# Autodesk Inventor assembly: FANUCs430
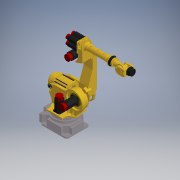
[picture p0: Inventor's stored thumbnail of the model, 180x180]
Saved by Autodesk Inventor 2017 (Build 210142000, 142)
## iProperties
Created: 2002-03-22
Part Number: FANUCs430
Document SubType Name: Assembly
Designer: sdotson
Control State: 0
Master: False
Checked Out: False
Shininess: 0.0
Length Units: 11269
Angle Units: 11279
Time Units: 11290
Mass Units: 11283
Length Display Precision: 3
Angle Display Precision: 2
Compacted: True
Density: 0.0
Volumn: 0.0
Area: 0.0
PropertySet Name: Model Information
Author: sdotson
## Documents named in this file (36)
- C:\Users\diego\Desktop\Example Inventor\12\toExporti.iam
- C:\Users\diego\Desktop\Example Inventor\12\s430if1.ipt
- C:\Users\diego\Desktop\Example Inventor\12\s430if13.ipt
- C:\Users\diego\Desktop\Example Inventor\12\s430if12.ipt
- C:\Users\diego\Desktop\Example Inventor\12\s430if10.ipt
- C:\Users\diego\Desktop\Example Inventor\12\s430if9.ipt
- C:\Users\diego\Desktop\Example Inventor\12\s430if14.ipt
- C:\Users\diego\Desktop\Example Inventor\12\s430if86.ipt
- C:\Users\diego\Desktop\Example Inventor\12\s430if85.ipt
- C:\Users\diego\Desktop\Example Inventor\12\s430if87.ipt
- C:\Users\diego\Desktop\Example Inventor\12\s430if88.ipt
- C:\Users\diego\Desktop\Example Inventor\12\s430if82.ipt
- C:\Users\diego\Desktop\Example Inventor\12\s430if83.ipt
- C:\Users\diego\Desktop\Example Inventor\12\s430if84.ipt
- C:\Users\diego\Desktop\Example Inventor\12\s430if34.ipt
- C:\Users\diego\Desktop\Example Inventor\12\s430if40.ipt
- C:\Users\diego\Desktop\Example Inventor\12\s430if63.ipt
- C:\Users\diego\Desktop\Example Inventor\12\NutPlate.iam
- C:\Users\diego\Desktop\Example Inventor\12\s430if24.ipt
- C:\Users\diego\Desktop\Example Inventor\12\NutPlate2.iam
- C:\Users\diego\Desktop\Example Inventor\12\s430if30.ipt
- C:\Users\diego\Desktop\Example Inventor\12\s430if31.ipt
- C:\Users\diego\Desktop\Example Inventor\12\s430if58.ipt
- C:\Users\diego\Desktop\Example Inventor\12\s430if57.ipt
- C:\Users\diego\Desktop\Example Inventor\12\s430if35.ipt
- C:\Users\diego\Desktop\Example Inventor\12\s430if59.ipt
- C:\Users\diego\Desktop\Example Inventor\12\s430if15.ipt
- C:\Users\diego\Desktop\Example Inventor\12\s430if74.ipt
- C:\Users\diego\Desktop\Example Inventor\12\SmallServo.iam
- C:\Users\diego\Desktop\Example Inventor\12\s430if23.ipt
- C:\Users\diego\Desktop\Example Inventor\12\s430if3.ipt
- C:\Users\diego\Desktop\Example Inventor\12\s430if22.ipt
- C:\Users\diego\Desktop\Example Inventor\12\s430if5.ipt
- C:\Users\diego\Desktop\Example Inventor\12\s430if6.ipt
- C:\Users\diego\Desktop\Example Inventor\12\AXIS5.ipt
- C:\Users\diego\Desktop\Example Inventor\12\AXIS6.ipt
## Components (50 placed, 35 different names)
1. s430if1:1 — Insertar:1, Ángulo:2, Nivelación:11, Nivelación:12, Coincidencia:37, Ángulo:13
2. s430if13:1 — Insertar:1, Insertar:2
3. s430if12:1 — Insertar:2, Insertar:3
4. s430if12:2 — Insertar:3, Insertar:4
5. s430if10:1 — Insertar:4, Insertar:5
6. s430if9:1 — Insertar:5, Coincidencia:1, Coincidencia:2
7. J1 — Coincidencia:1, Coincidencia:2, Coincidencia:3, Nivelación:1, Coincidencia:4, Insertar:6, Insertar:15, Insertar:16, Coincidencia:16, Insertar:17, Insertar:18, Coincidencia:17, Coincidencia:18, Insertar:19, Coincidencia:19, Coincidencia:20, Nivelación:3, Insertar:22, Ángulo:12
8. s430if86:1 — Coincidencia:3, Nivelación:1, Coincidencia:4, Nivelación:2, Coincidencia:5, Coincidencia:6
9. s430if85:1 — Nivelación:2, Coincidencia:5, Coincidencia:6, Coincidencia:7, Coincidencia:8, Ángulo:1
10. s430if87:1 — Coincidencia:7, Coincidencia:8, Ángulo:1
11. s430if88:1 — Coincidencia:12, Coincidencia:14, Ángulo:4
12. s430if82:1 — Coincidencia:11, Coincidencia:13, Coincidencia:14, Ángulo:3, Ángulo:4
13. s430if83:1 — Coincidencia:9, Coincidencia:10, Ángulo:2, Coincidencia:11, Coincidencia:12, Coincidencia:13, Ángulo:3
14. s430if84:1 — Insertar:6, Coincidencia:9, Coincidencia:10
15. s430if34:1 — Insertar:7, Insertar:8, Insertar:9, Insertar:10, Insertar:11, Insertar:12, Insertar:13, Insertar:14, Coincidencia:15, Coincidencia:16, Ángulo:11, Coincidencia:38
16. s430if40:1 — Insertar:7
17. s430if40:2 — Insertar:8
18. s430if40:3 — Insertar:10
19. s430if40:4 — Insertar:9
20. s430if40:5 — Insertar:11
21. s430if40:6 — Insertar:12
22. s430if40:7 — Insertar:13
23. s430if40:8 — Insertar:14
24. s430if63:1 — Insertar:15, Coincidencia:15
25. s430if63:2 — Insertar:16
26. NutPlate:1 [sub-assembly] — Insertar:18
27. NutPlate:2 [sub-assembly] — Insertar:17
28. J2 — Coincidencia:17, Coincidencia:18, Coincidencia:24, Insertar:23, Insertar:24, Ángulo:13, Ángulo:14
29. NutPlate2:1 [sub-assembly] — Insertar:19
30. s430if30:1 — Coincidencia:19, Coincidencia:20, Nivelación:3, Coincidencia:21, Coincidencia:22
31. s430if31:1 — Coincidencia:21, Coincidencia:22
32. s430if58:1 — Coincidencia:23, Insertar:21, Coincidencia:24
33. s430if57:1 — Coincidencia:23, Insertar:20, Insertar:21
34. s430if35:1 — Insertar:20, Ángulo:11, Coincidencia:38
35. s430if59:1 — Insertar:22
36. J3 — Insertar:23, Coincidencia:25, Coincidencia:26, Ángulo:5, Coincidencia:27, Coincidencia:29, Coincidencia:31, Nivelación:4, Nivelación:5, Coincidencia:32, Coincidencia:33, Nivelación:8, Nivelación:9, Insertar:25, Ángulo:10, Ángulo:14
37. s430if74:1 — Insertar:24
38. s430if86:2 — Coincidencia:25, Coincidencia:26, Ángulo:5, Coincidencia:28, Ángulo:7
39. s430if85:2 — Coincidencia:27, Coincidencia:28, Coincidencia:30, Ángulo:6, Ángulo:7
40. s430if87:2 — Coincidencia:29, Coincidencia:30, Ángulo:6
41. SmallServo:1 [sub-assembly] — Coincidencia:31, Nivelación:4, Nivelación:5, Ángulo:8, Nivelación:7
42. SmallServo:2 [sub-assembly] — Coincidencia:32, Ángulo:8, Ángulo:9, Nivelación:6, Nivelación:7, Nivelación:8
43. SmallServo:3 [sub-assembly] — Coincidencia:33, Ángulo:9, Nivelación:6, Nivelación:9
44. s430if23:1 — Insertar:25, Ángulo:10, Insertar:26, Ángulo:15
45. s430if3:1 — Insertar:26, Insertar:27
46. J4 — Insertar:27, Coincidencia:34, Coincidencia:35, Coincidencia:36, Nivelación:10, Ángulo:15, Ángulo:16
47. s430if5:1 — Coincidencia:34, Insertar:28, Insertar:29
48. s430if6:1 — Coincidencia:35, Insertar:29
49. J5 — Coincidencia:36, Nivelación:10, Insertar:28, Insertar:30, Angle, Ángulo:16
50. J6 — Insertar:30, Angle
## Relationships (97: Mate 38, Insert 30, Angle 17, Flush 12)
- Insertar:1: s430if1:1 ↔ s430if13:1
- Insertar:2: s430if13:1 ↔ s430if12:1
- Insertar:3: s430if12:1 ↔ s430if12:2
- Insertar:4: s430if12:2 ↔ s430if10:1
- Insertar:5: s430if10:1 ↔ s430if9:1
- Coincidencia:1 [Mate]: s430if9:1 ↔ J1
- Coincidencia:2 [Mate]: s430if9:1 ↔ J1
- Coincidencia:3 [Mate]: J1 ↔ s430if86:1
- Nivelación:1 [Flush] (117.314 mm): J1 ↔ s430if86:1
- Coincidencia:4 [Mate]: J1 ↔ s430if86:1
- Nivelación:2 [Flush]: s430if86:1 ↔ s430if85:1
- Coincidencia:5 [Mate]: s430if86:1 ↔ s430if85:1
- Coincidencia:6 [Mate]: s430if86:1 ↔ s430if85:1
- Coincidencia:7 [Mate]: s430if85:1 ↔ s430if87:1
- Coincidencia:8 [Mate]: s430if85:1 ↔ s430if87:1
- Ángulo:1 [Angle] (0 deg): s430if85:1 ↔ s430if87:1
- Insertar:6: J1 ↔ s430if84:1
- Coincidencia:9 [Mate]: s430if83:1 ↔ s430if84:1
- Coincidencia:10 [Mate]: s430if83:1 ↔ s430if84:1
- Ángulo:2 [Angle] (0 deg): s430if1:1 ↔ s430if83:1
- Coincidencia:11 [Mate]: s430if82:1 ↔ s430if83:1
- Coincidencia:12 [Mate]: s430if88:1 ↔ s430if83:1
- Coincidencia:13 [Mate]: s430if82:1 ↔ s430if83:1
- Coincidencia:14 [Mate]: s430if88:1 ↔ s430if82:1
- Ángulo:3 [Angle] (0 deg): s430if82:1 ↔ s430if83:1
- Ángulo:4 [Angle] (0 deg): s430if88:1 ↔ s430if82:1
- Insertar:7: s430if34:1 ↔ s430if40:1
- Insertar:8: s430if34:1 ↔ s430if40:2
- Insertar:9: s430if34:1 ↔ s430if40:4
- Insertar:10: s430if34:1 ↔ s430if40:3
- Insertar:11: s430if34:1 ↔ s430if40:5
- Insertar:12: s430if34:1 ↔ s430if40:6
- Insertar:13: s430if34:1 ↔ s430if40:7
- Insertar:14: s430if34:1 ↔ s430if40:8
- Insertar:15: J1 ↔ s430if63:1
- Insertar:16: J1 ↔ s430if63:2
- Coincidencia:15 [Mate]: s430if34:1 ↔ s430if63:1
- Coincidencia:16 [Mate] (16.276 mm): J1 ↔ s430if34:1
- Insertar:17: J1 ↔ NutPlate:2
- Insertar:18: J1 ↔ NutPlate:1
- Coincidencia:17 [Mate]: J1 ↔ J2
- Coincidencia:18 [Mate] (17.998 mm): J1 ↔ J2
- Insertar:19: J1 ↔ NutPlate2:1
- Coincidencia:19 [Mate]: J1 ↔ s430if30:1
- Coincidencia:20 [Mate]: J1 ↔ s430if30:1
- Nivelación:3 [Flush]: J1 ↔ s430if30:1
- Coincidencia:21 [Mate]: s430if30:1 ↔ s430if31:1
- Coincidencia:22 [Mate]: s430if30:1 ↔ s430if31:1
- Coincidencia:23 [Mate]: s430if58:1 ↔ s430if57:1
- Insertar:20: s430if57:1 ↔ s430if35:1
- Insertar:21: s430if58:1 ↔ s430if57:1
- Coincidencia:24 [Mate]: J2 ↔ s430if58:1
- Insertar:22: J1 ↔ s430if59:1
- Insertar:23: J2 ↔ J3
- Insertar:24: J2 ↔ s430if74:1
- Coincidencia:25 [Mate]: J3 ↔ s430if86:2
- Coincidencia:26 [Mate]: J3 ↔ s430if86:2
- Ángulo:5 [Angle] (0 deg): J3 ↔ s430if86:2
- Coincidencia:27 [Mate]: J3 ↔ s430if85:2
- Coincidencia:28 [Mate]: s430if86:2 ↔ s430if85:2
- Coincidencia:29 [Mate]: J3 ↔ s430if87:2
- Coincidencia:30 [Mate]: s430if85:2 ↔ s430if87:2
- Ángulo:6 [Angle] (0 deg): s430if85:2 ↔ s430if87:2
- Ángulo:7 [Angle] (0 deg): s430if86:2 ↔ s430if85:2
- Coincidencia:31 [Mate]: J3 ↔ SmallServo:1
- Nivelación:4 [Flush] (7.881 mm): J3 ↔ SmallServo:1
- Nivelación:5 [Flush] (9.824 mm): J3 ↔ SmallServo:1
- Coincidencia:32 [Mate]: J3 ↔ SmallServo:2
- Coincidencia:33 [Mate]: J3 ↔ SmallServo:3
- Ángulo:8 [Angle] (0 deg): SmallServo:1 ↔ SmallServo:2
- Ángulo:9 [Angle] (0 deg): SmallServo:2 ↔ SmallServo:3
- Nivelación:6 [Flush]: SmallServo:2 ↔ SmallServo:3
- Nivelación:7 [Flush]: SmallServo:1 ↔ SmallServo:2
- Nivelación:8 [Flush] (3.8 mm): J3 ↔ SmallServo:2
- Nivelación:9 [Flush] (4.924 mm): J3 ↔ SmallServo:3
- Insertar:25: J3 ↔ s430if23:1
- Ángulo:10 [Angle] (0 deg): J3 ↔ s430if23:1
- Insertar:26: s430if23:1 ↔ s430if3:1
- Insertar:27: s430if3:1 ↔ J4
- Coincidencia:34 [Mate]: J4 ↔ s430if5:1
- Coincidencia:35 [Mate]: J4 ↔ s430if6:1
- Coincidencia:36 [Mate]: J4 ↔ J5
- Nivelación:10 [Flush]: J4 ↔ J5
- Insertar:28: s430if5:1 ↔ J5
- Insertar:29: s430if5:1 ↔ s430if6:1
- Insertar:30: J5 ↔ J6
- Nivelación:11 [Flush]: s430if1:1
- Nivelación:12 [Flush]: s430if1:1
- Coincidencia:37 [Mate]: s430if1:1
- Ángulo:11 [Angle] (0 deg): s430if34:1 ↔ s430if35:1
- Coincidencia:38 [Mate]: s430if34:1 ↔ s430if35:1
- Ángulo:12 [Angle] (0 deg): J1
- Ángulo:13 [Angle] (0 deg): s430if1:1 ↔ J2
- Ángulo:14 [Angle] (0 deg): J2 ↔ J3
- Ángulo:15 [Angle] (0 deg): s430if23:1 ↔ J4
- Angle (0 deg): J5 ↔ J6
- Ángulo:16 [Angle] (0 deg): J4 ↔ J5
## Named parameters: J1 = 0 deg, J2 = 0 deg, J3 = 0 deg, J4 = 0 deg, J5 = 0 deg, J6 = 0 deg
